# Autodesk Inventor assembly: Assembly1
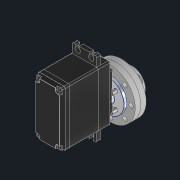
[picture p0: Inventor's stored thumbnail of the model, 180x180]
Saved by Autodesk Inventor 2022 (Build 260153000, 153)
## iProperties
Created: 2021-08-27
Part Number: Assembly1
Document SubType Name: Assembly
Designer: Yuta Kage
Author: Yuta Kage
## Documents named in this file (6)
- C:\Users\yuta0\Documents\GitHub\catchrobo_hardware\assy-shooter\Assembly1.iam
- C:\Users\yuta0\Documents\GitHub\catchrobo_hardware\assy-robot\MG_996R.iam
- C:\Users\yuta0\Documents\GitHub\catchrobo_hardware\assy-shooter\s_base5.ipt
- C:\Users\yuta0\Documents\GitHub\catchrobo_hardware\assy-robot\CB3-10.ipt
- C:\Users\yuta0\Documents\GitHub\catchrobo_hardware\assy-shooter\s_base6.ipt
- C:\Users\yuta0\Documents\GitHub\catchrobo_hardware\assy-shooter\SCSTR6-8.iam
## Components (12 placed, 5 different names)
1. MG_996R:1 [sub-assembly] — メイト:1, メイト:2, メイト:3
2. s_base5:1 — メイト:1, メイト:2, メイト:3, メイト:4, メイト:5, メイト:9, メイト:13
3. s_base6:1 — メイト:6, メイト:7, メイト:8, メイト:9, メイト:10, メイト:11, メイト:12, メイト:13
4. SCSTR6-8:1 [sub-assembly] — メイト:6, メイト:7, メイト:8
5. CB3-10:1 — メイト:4, メイト:5
6. CB3-10:5 — メイト:11, メイト:12
7. CB3-10:2
8. CB3-10:6
9. CB3-10:3
10. CB3-10:7
11. CB3-10:4 — メイト:10
12. CB3-10:8
## Component patterns: (4 elements, first: CB3-10:1 + CB3-10:5)
## Relationships (13: Mate 13)
- メイト:1 [Mate]: MG_996R:1 ↔ s_base5:1
- メイト:2 [Mate]: MG_996R:1 ↔ s_base5:1
- メイト:3 [Mate]: MG_996R:1 ↔ s_base5:1
- メイト:4 [Mate]: s_base5:1 ↔ CB3-10:1
- メイト:5 [Mate]: s_base5:1 ↔ CB3-10:1
- メイト:6 [Mate]: s_base6:1 ↔ SCSTR6-8:1
- メイト:7 [Mate]: s_base6:1 ↔ SCSTR6-8:1
- メイト:8 [Mate]: s_base6:1 ↔ SCSTR6-8:1
- メイト:9 [Mate]: s_base5:1 ↔ s_base6:1
- メイト:10 [Mate]: s_base6:1 ↔ CB3-10:4
- メイト:11 [Mate]: s_base6:1 ↔ CB3-10:5
- メイト:12 [Mate]: s_base6:1 ↔ CB3-10:5
- メイト:13 [Mate]: s_base5:1 ↔ s_base6:1
